# Autodesk Inventor assembly: Kühler_vorne
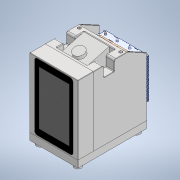
[picture p0: Inventor's stored thumbnail of the model, 180x180]
Saved by Autodesk Inventor 2021 (Build 250183000, 183)
## iProperties
Created: 2021-07-20
Part Number: Kühler_vorne
Document SubType Name: Assembly
Designer: Simon
Author: Simon
## Documents named in this file (11)
- C:\WORK\MILK_COOLER\Kühler_vorne.iam
- C:\WORK\MILK_COOLER\display_halter.ipt
- C:\WORK\MILK_COOLER\display_mit_pi.iam
- C:\WORK\MILK_COOLER\milch_halter.ipt
- C:\WORK\MILK_COOLER\milch.ipt
- C:\WORK\MILK_COOLER\kühlblock.ipt
- C:\WORK\MILK_COOLER\peltier.ipt
- C:\WORK\MILK_COOLER\Noctua-NH-L12S.iam
- C:\WORK\MILK_COOLER\Noctua NF-A12x15.ipt
- C:\WORK\MILK_COOLER\magnet.ipt
- C:\WORK\MILK_COOLER\boden.ipt
## Components (27 placed, 10 different names)
1. display_halter:1 — Fluchtend:1, Fluchtend:2, Fluchtend:3, Passend:1, Passend:2, Passend:3, Fluchtend:4, Einfügen:1, Einfügen:2, Einfügen:3, Einfügen:4, Fluchtend:8, Einfügen:15, Einfügen:16, Passend:20, Passend:21
2. display_mit_pi:1 [sub-assembly] — Passend:1, Passend:2, Passend:3
3. milch_halter:1 — Fluchtend:4, Passend:4, Passend:5, Passend:7, Passend:17, Einfügen:5, Einfügen:6, Einfügen:7, Einfügen:8, Einfügen:9, Einfügen:10, Fluchtend:9, Passend:19, Einfügen:17, Einfügen:18, Passend:21, Passend:22
4. milch:1 — Passend:4, Passend:5
5. kühlblock:1 — Passend:7, Passend:11, Passend:12, Passend:13, Passend:17, Passend:19
6. peltier:1 — Passend:8, Passend:9, Passend:10, Passend:13
7. Noctua-NH-L12S:1 [sub-assembly] — Passend:8, Passend:9, Passend:10, Passend:11, Passend:12, Passend:14, Passend:15, Fluchtend:7
8. Noctua NF-A12x15:1 — Passend:14, Passend:15, Fluchtend:7
9. magnet:1 — Einfügen:2
10. magnet:2 — Einfügen:4
11. magnet:3 — Einfügen:1
12. magnet:4 — Einfügen:3
13. magnet:5 — Einfügen:8
14. magnet:6 — Einfügen:7
15. magnet:7 — Einfügen:6
16. magnet:8 — Einfügen:5
17. magnet:9 — Einfügen:10
18. magnet:10 — Einfügen:9
19. boden:1 — Fluchtend:8, Fluchtend:9, Einfügen:11, Einfügen:12, Einfügen:13, Einfügen:14, Passend:20, Passend:22
20. magnet:11 — Einfügen:11
21. magnet:12 — Einfügen:13
22. magnet:13 — Einfügen:14
23. magnet:14 — Einfügen:15
24. magnet:15 — Einfügen:12
25. magnet:16 — Einfügen:18
26. magnet:17 — Einfügen:17
27. magnet:18 — Einfügen:16
## Relationships (44: Mate 19, Insert 18, Flush 7)
- Fluchtend:1 [Flush]: display_halter:1
- Fluchtend:2 [Flush]: display_halter:1
- Fluchtend:3 [Flush]: display_halter:1
- Passend:1 [Mate] (0.5 mm): display_halter:1 ↔ display_mit_pi:1
- Passend:2 [Mate] (0.5 mm): display_halter:1 ↔ display_mit_pi:1
- Passend:3 [Mate]: display_halter:1 ↔ display_mit_pi:1
- Fluchtend:4 [Flush]: display_halter:1 ↔ milch_halter:1
- Passend:4 [Mate] (7.5 mm): milch_halter:1 ↔ milch:1
- Passend:5 [Mate]: milch_halter:1 ↔ milch:1
- Passend:7 [Mate] (1 mm): milch_halter:1 ↔ kühlblock:1
- Passend:8 [Mate]: peltier:1 ↔ Noctua-NH-L12S:1
- Passend:9 [Mate] (2.5 mm): peltier:1 ↔ Noctua-NH-L12S:1
- Passend:10 [Mate]: peltier:1 ↔ Noctua-NH-L12S:1
- Passend:11 [Mate]: kühlblock:1 ↔ Noctua-NH-L12S:1
- Passend:12 [Mate]: kühlblock:1 ↔ Noctua-NH-L12S:1
- Passend:13 [Mate]: kühlblock:1 ↔ peltier:1
- Passend:14 [Mate]: Noctua-NH-L12S:1 ↔ Noctua NF-A12x15:1
- Passend:15 [Mate] (1 mm): Noctua-NH-L12S:1 ↔ Noctua NF-A12x15:1
- Fluchtend:7 [Flush] (4 mm): Noctua-NH-L12S:1 ↔ Noctua NF-A12x15:1
- Passend:17 [Mate]: milch_halter:1 ↔ kühlblock:1
- Einfügen:1 [Insert]: display_halter:1 ↔ magnet:3
- Einfügen:2 [Insert]: display_halter:1 ↔ magnet:1
- Einfügen:3 [Insert]: display_halter:1 ↔ magnet:4
- Einfügen:4 [Insert]: display_halter:1 ↔ magnet:2
- Einfügen:5 [Insert]: milch_halter:1 ↔ magnet:8
- Einfügen:6 [Insert]: milch_halter:1 ↔ magnet:7
- Einfügen:7 [Insert]: milch_halter:1 ↔ magnet:6
- Einfügen:8 [Insert]: milch_halter:1 ↔ magnet:5
- Einfügen:9 [Insert]: milch_halter:1 ↔ magnet:10
- Einfügen:10 [Insert]: milch_halter:1 ↔ magnet:9
- Fluchtend:8 [Flush]: display_halter:1 ↔ boden:1
- Fluchtend:9 [Flush]: milch_halter:1 ↔ boden:1
- Passend:19 [Mate]: milch_halter:1 ↔ kühlblock:1
- Einfügen:11 [Insert]: boden:1 ↔ magnet:11
- Einfügen:12 [Insert]: boden:1 ↔ magnet:15
- Einfügen:13 [Insert]: boden:1 ↔ magnet:12
- Einfügen:14 [Insert]: boden:1 ↔ magnet:13
- Einfügen:15 [Insert]: display_halter:1 ↔ magnet:14
- Einfügen:16 [Insert]: display_halter:1 ↔ magnet:18
- Einfügen:17 [Insert]: milch_halter:1 ↔ magnet:17
- Einfügen:18 [Insert]: milch_halter:1 ↔ magnet:16
- Passend:20 [Mate]: display_halter:1 ↔ boden:1
- Passend:21 [Mate]: display_halter:1 ↔ milch_halter:1
- Passend:22 [Mate]: milch_halter:1 ↔ boden:1
